# Autodesk Inventor assembly: main_assembly
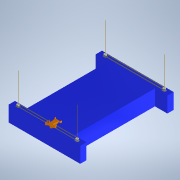
[picture p0: Inventor's stored thumbnail of the model, 180x180]
Saved by Autodesk Inventor 2020 (Build 240168000, 168)
## iProperties
Created: 2021-03-06
Part Number: main_assembly
Document SubType Name: Assembly
Designer: Harry
Author: Harry
## Documents named in this file (8)
- C:\Users\Harry\Documents\hacktheburgh\octocatch\cad\main_assembly.iam
- C:\Users\Harry\Documents\hacktheburgh\octocatch\cad\backplate.ipt
- C:\Users\Harry\Documents\hacktheburgh\octocatch\cad\dc_motor_larger.ipt
- C:\Users\Harry\Documents\hacktheburgh\octocatch\cad\belt_gear.ipt
- C:\Users\Harry\Documents\hacktheburgh\octocatch\cad\main_assembly\Design Accelerator\Synchronous Belts Transmission1.iam
- C:\Users\Harry\Documents\hacktheburgh\octocatch\cad\octopus_on_belt.ipt
- C:\Users\Harry\Documents\hacktheburgh\octocatch\cad\large_motor_with_gear.iam
- C:\Users\Harry\Documents\hacktheburgh\octocatch\cad\main_assembly\Design Accelerator\Synchronous Belts Transmission2.iam
## Components (10 placed, 6 different names)
1. backplate:1 — Insert:1, Insert:2, Insert:5, Insert:6
2. dc_motor_larger:1 — Insert:1, Insert:3
3. dc_motor_larger:2 — Insert:2, Insert:4
4. belt_gear:1 — Insert:3
5. belt_gear:2 — Insert:4
6. Synchronous Belts Transmission:1 [sub-assembly] — Mate:1, Mate:2
7. octopus_on_belt:1 — Mate:1, Mate:2
8. large_motor_with_gear:1 [sub-assembly] — Insert:5
9. large_motor_with_gear:2 [sub-assembly] — Insert:6
10. Synchronous Belts Transmission:2 [sub-assembly]
## Relationships (8: Insert 6, Mate 2)
- Insert:1: backplate:1 ↔ dc_motor_larger:1
- Insert:2: backplate:1 ↔ dc_motor_larger:2
- Insert:3: dc_motor_larger:1 ↔ belt_gear:1
- Insert:4: dc_motor_larger:2 ↔ belt_gear:2
- Mate:1: Synchronous Belts Transmission:1 ↔ octopus_on_belt:1
- Mate:2: Synchronous Belts Transmission:1 ↔ octopus_on_belt:1
- Insert:5: backplate:1 ↔ large_motor_with_gear:1
- Insert:6: backplate:1 ↔ large_motor_with_gear:2
